# Autodesk Inventor assembly: Assembly-9V Holder
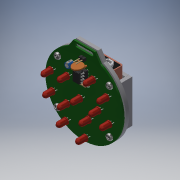
[picture p0: Inventor's stored thumbnail of the model, 180x180]
Saved by Autodesk Inventor 2018.3 (Build 223284000, 284)
## iProperties
Created: 2019-07-21
Part Number: Assembly-9V Holder
Document SubType Name: Assembly
Designer: Electro707
Author: Electro707
## Documents named in this file (5)
- F:\Projects\UNH MakerSpace Kits\2019 - Winter Holiday\Ornament\GitHub Folder\CAD - Inventor\Assembly-9V Holder.iam
- F:\Projects\UNH MakerSpace Kits\2019 - Winter Holiday\Ornament\GitHub Folder\CAD - Inventor\ANSI B18.6.7M - M3x0.5 x 6(4).ipt
- F:\Projects\UNH MakerSpace Kits\2019 - Winter Holiday\Ornament\GitHub Folder\CAD - Inventor\Assembly-PCB alone.iam
- F:\Projects\UNH MakerSpace Kits\2019 - Winter Holiday\Ornament\GitHub Folder\CAD - Inventor\Back Plate - 9V.iam
- F:\Projects\UNH MakerSpace Kits\2019 - Winter Holiday\Ornament\GitHub Folder\CAD - Inventor\9V Battery.ipt
## Components (7 placed, 4 different names)
1. ANSI B18.6.7M - M3x0.5 x 6(4):7 — Mate:21, Mate:24
2. ANSI B18.6.7M - M3x0.5 x 6(4):8 — Mate:19, Mate:23, Flush:1
3. ANSI B18.6.7M - M3x0.5 x 6(4):9 — Mate:17, Mate:22
4. ANSI B18.6.7M - M3x0.5 x 6(4):10 — Mate:16, Mate:20, Mate:18
5. Assembly-PCB alone:1 [sub-assembly] — Mate:16, Mate:17, Mate:19, Mate:20, Mate:21, Mate:22, Mate:23, Mate:25, Mate:24
6. Back Plate - 9V:2 [sub-assembly] — Flush:1, Mate:26, Mate:27, Mate:28, Mate:32, Angle:5, Mate:18, Mate:25
7. 9V Battery:1 — Mate:26, Mate:29, Angle:3, Mate:31, Angle:4
## Relationships (25: Mate 18, Angle 5, Flush 1, Symmetry 1)
- Mate:16: ANSI B18.6.7M - M3x0.5 x 6(4):10 ↔ Assembly-PCB alone:1
- Mate:17: ANSI B18.6.7M - M3x0.5 x 6(4):9 ↔ Assembly-PCB alone:1
- Mate:18: ANSI B18.6.7M - M3x0.5 x 6(4):10 ↔ Back Plate - 9V:2
- Mate:19: ANSI B18.6.7M - M3x0.5 x 6(4):8 ↔ Assembly-PCB alone:1
- Mate:20: ANSI B18.6.7M - M3x0.5 x 6(4):10 ↔ Assembly-PCB alone:1
- Mate:21: ANSI B18.6.7M - M3x0.5 x 6(4):7 ↔ Assembly-PCB alone:1
- Mate:22: ANSI B18.6.7M - M3x0.5 x 6(4):9 ↔ Assembly-PCB alone:1
- Mate:23: ANSI B18.6.7M - M3x0.5 x 6(4):8 ↔ Assembly-PCB alone:1
- Mate:24: ANSI B18.6.7M - M3x0.5 x 6(4):7 ↔ Assembly-PCB alone:1
- Mate:25: Assembly-PCB alone:1 ↔ Back Plate - 9V:2
- Flush:1: ANSI B18.6.7M - M3x0.5 x 6(4):8 ↔ Back Plate - 9V:2
- Mate:26: Back Plate - 9V:2 ↔ 9V Battery:1
- Mate:27: Back Plate - 9V:2
- Angle:1 (0 deg)
- Mate:28: Back Plate - 9V:2
- Angle:2 (0 deg)
- Symmetry:1
- Mate:29: 9V Battery:1
- Angle:3 (0 deg): 9V Battery:1
- Mate:30
- Mate:31: 9V Battery:1
- Angle:4 (0 deg): 9V Battery:1
- Mate:32: Back Plate - 9V:2
- Angle:5 (0 deg): Back Plate - 9V:2
- Mate:33
